# Autodesk Inventor assembly: chaimber
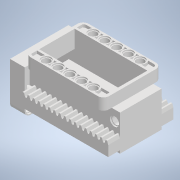
[picture p0: Inventor's stored thumbnail of the model, 180x180]
Saved by Autodesk Inventor 2021 (Build 250183000, 183)
## iProperties
Created: 2024-03-14
Part Number: chaimber
Document SubType Name: Assembly
Designer: 22hamfri
Author: 22hamfri
## Documents named in this file (6)
- C:\Users\22hamfri\Documents\School\Programmering\domino-bil\CAD\chaimber.iam
- C:\Users\22hamfri\Documents\School\Programmering\domino-bil\CAD\chaimber.ipt
- C:\Users\22hamfri\Documents\School\Programmering\domino-bil\CAD\chaimber-adapter.ipt
- C:\Users\22hamfri\Documents\School\Programmering\domino-bil\CAD\magazine-adapter.ipt
- C:\Users\22hamfri\Documents\School\Programmering\domino-bil\CAD\chaimber-bolt.ipt
- C:\Users\22hamfri\Documents\School\Programmering\domino-bil\CAD\bolt-rack.ipt
## Components (6 placed, 5 different names)
1. chaimber:1 — Rigid:1, Rigid:2, Angle:1, Mate:1, bolt-action
2. chaimber-adapter:1 — Rigid:1
3. magazine-adapter:1 — Rigid:2
4. chaimber-bolt:1 — Angle:1, Mate:1, bolt-action, Rigid:3, Rigid:4
5. bolt-rack:1 — Rigid:3
6. bolt-rack:2 — Rigid:4
## Relationships (7: WeldJoint 4, Mate 2, Angle 1)
- Rigid:1 [WeldJoint]: chaimber:1 ↔ chaimber-adapter:1
- Rigid:2 [WeldJoint]: chaimber:1 ↔ magazine-adapter:1
- Angle:1 (180 deg): chaimber:1 ↔ chaimber-bolt:1
- Mate:1: chaimber:1 ↔ chaimber-bolt:1
- bolt-action [Mate]: chaimber:1 ↔ chaimber-bolt:1
- Rigid:3 [WeldJoint]: chaimber-bolt:1 ↔ bolt-rack:1
- Rigid:4 [WeldJoint]: chaimber-bolt:1 ↔ bolt-rack:2
